# Autodesk Inventor assembly: assembly
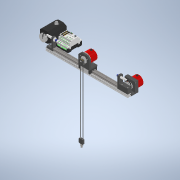
[picture p0: Inventor's stored thumbnail of the model, 180x180]
Saved by Autodesk Inventor 2021 (Build 250183000, 183)
## iProperties
Created: 2022-07-01
Part Number: assembly
Document SubType Name: Assembly
Designer: lenna
Author: lenna
## Documents named in this file (4)
- C:\Users\lenna\Desktop\Lennart\Uni\Master\2. Semester\SDM\CAD_neu\assembly.iam
- C:\Users\lenna\Desktop\Lennart\Uni\Master\2. Semester\SDM\CAD_neu\base_assembly.iam
- C:\Users\lenna\Desktop\Lennart\Uni\Master\2. Semester\SDM\CAD_neu\cart_assembly.iam
- C:\Users\lenna\Desktop\Lennart\Uni\Master\2. Semester\SDM\CAD_neu\pendulum_assembly.iam
## Components (3 placed, 3 different names)
1. base_assembly:1 [sub-assembly] — Mate:1, Flush:1, Flush:2, Mate:2, Mate:3
2. cart_assembly:1 [sub-assembly] — Mate:2, Mate:3, Insert:1, Angle:1
3. pendulum_assembly:1 [sub-assembly] — Insert:1, Angle:1
## Relationships (7: Mate 3, Flush 2, Insert 1, Angle 1)
- Mate:1: base_assembly:1
- Flush:1: base_assembly:1
- Flush:2: base_assembly:1
- Mate:2: base_assembly:1 ↔ cart_assembly:1
- Mate:3: base_assembly:1 ↔ cart_assembly:1
- Insert:1: cart_assembly:1 ↔ pendulum_assembly:1
- Angle:1 (180 deg): cart_assembly:1 ↔ pendulum_assembly:1
